# Autodesk Inventor assembly: Sestava_kamera_static
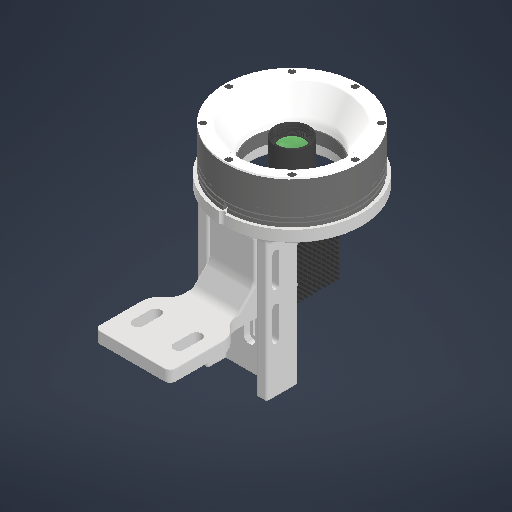
[picture p0: Inventor's stored thumbnail of the model, 512x512]
Saved by Autodesk Inventor 2026 (Build 300175000, 175)
## iProperties
Created: 2025-04-25
Part Number: Sestava_kamera_static
Document SubType Name: Assembly
Designer: lisnik
Author: lisnik
## Documents named in this file (7)
- C:\Users\lisnik\OneDrive - JIC\Dokumenty\visual_inspection_cell_4\skripty\github\visual_inspection_cell_project\models\ipt_iam\Sestava_kamera_static.iam
- C:\Users\lisnik\OneDrive - JIC\Dokumenty\visual_inspection_cell_4\skripty\github\visual_inspection_cell_project\models\ipt_iam\ChladicAceU_M8_UNC_ST\ChladicAceU_M8_UNC_ST\ChladicAceU_M8_UNC_ST.iam
- C:\Users\lisnik\OneDrive - JIC\Dokumenty\visual_inspection_cell_4\skripty\github\visual_inspection_cell_project\models\ipt_iam\M1228-MPW3_210322\M1228-MPW3_210322.iam
- C:\Users\lisnik\OneDrive - JIC\Dokumenty\visual_inspection_cell_4\skripty\github\visual_inspection_cell_project\models\ipt_iam\VMR-11566W\VMR-11566W.iam
- C:\Users\lisnik\OneDrive - JIC\Dokumenty\visual_inspection_cell_4\skripty\github\visual_inspection_cell_project\models\ipt_iam\Basler ace 2 GigE.ipt
- C:\Users\lisnik\OneDrive - JIC\Dokumenty\visual_inspection_cell_4\skripty\github\visual_inspection_cell_project\models\ipt_iam\drzak_kamera_static_1.ipt
- C:\Users\lisnik\OneDrive - JIC\Dokumenty\visual_inspection_cell_4\skripty\github\visual_inspection_cell_project\models\ipt_iam\Drzak_svetlo_VMR_11566W_v2.ipt
## Components (6 placed, 6 different names)
1. ChladicAceU_M8_UNC_ST:1 [sub-assembly] — Proti sobě:6, Proti sobě:7, Proti sobě:8, Proti sobě:9, Proti sobě:10, Proti sobě:11, Proti sobě:12, Proti sobě:13
2. M1228-MPW3_210322:1 [sub-assembly] — Proti sobě:4, Proti sobě:5, Proti sobě:14
3. VMR-11566W:1 [sub-assembly] — Proti sobě:1, Proti sobě:2, Proti sobě:3
4. Basler ace 2 GigE:1 — Proti sobě:4, Proti sobě:5, Proti sobě:6, Proti sobě:7, Proti sobě:8, Proti sobě:9, Proti sobě:10, Proti sobě:14
5. drzak_kamera_static_1:1 — Proti sobě:15, Proti sobě:16, Proti sobě:17, Proti sobě:18, Proti sobě:19, Proti sobě:20
6. Drzak_svetlo_VMR_11566W_v2:1 — Proti sobě:1, Proti sobě:2, Proti sobě:3, Proti sobě:11, Proti sobě:12, Proti sobě:13, Proti sobě:15, Proti sobě:16, Proti sobě:17
## Relationships (20: Mate 20)
- Proti sobě:1 [Mate]: VMR-11566W:1 ↔ Drzak_svetlo_VMR_11566W_v2:1
- Proti sobě:2 [Mate]: VMR-11566W:1 ↔ Drzak_svetlo_VMR_11566W_v2:1
- Proti sobě:3 [Mate]: VMR-11566W:1 ↔ Drzak_svetlo_VMR_11566W_v2:1
- Proti sobě:4 [Mate]: M1228-MPW3_210322:1 ↔ Basler ace 2 GigE:1
- Proti sobě:5 [Mate]: M1228-MPW3_210322:1 ↔ Basler ace 2 GigE:1
- Proti sobě:6 [Mate]: ChladicAceU_M8_UNC_ST:1 ↔ Basler ace 2 GigE:1
- Proti sobě:7 [Mate]: ChladicAceU_M8_UNC_ST:1 ↔ Basler ace 2 GigE:1
- Proti sobě:8 [Mate]: ChladicAceU_M8_UNC_ST:1 ↔ Basler ace 2 GigE:1
- Proti sobě:9 [Mate]: ChladicAceU_M8_UNC_ST:1 ↔ Basler ace 2 GigE:1
- Proti sobě:10 [Mate]: ChladicAceU_M8_UNC_ST:1 ↔ Basler ace 2 GigE:1
- Proti sobě:11 [Mate]: ChladicAceU_M8_UNC_ST:1 ↔ Drzak_svetlo_VMR_11566W_v2:1
- Proti sobě:12 [Mate]: ChladicAceU_M8_UNC_ST:1 ↔ Drzak_svetlo_VMR_11566W_v2:1
- Proti sobě:13 [Mate]: ChladicAceU_M8_UNC_ST:1 ↔ Drzak_svetlo_VMR_11566W_v2:1
- Proti sobě:14 [Mate]: M1228-MPW3_210322:1 ↔ Basler ace 2 GigE:1
- Proti sobě:15 [Mate]: drzak_kamera_static_1:1 ↔ Drzak_svetlo_VMR_11566W_v2:1
- Proti sobě:16 [Mate]: drzak_kamera_static_1:1 ↔ Drzak_svetlo_VMR_11566W_v2:1
- Proti sobě:17 [Mate]: drzak_kamera_static_1:1 ↔ Drzak_svetlo_VMR_11566W_v2:1
- Proti sobě:18 [Mate]: drzak_kamera_static_1:1
- Proti sobě:19 [Mate]: drzak_kamera_static_1:1
- Proti sobě:20 [Mate]: drzak_kamera_static_1:1
